# Autodesk Inventor assembly: Folded Door with the Rollers
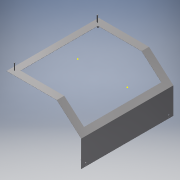
[picture p0: Inventor's stored thumbnail of the model, 180x180]
Saved by Autodesk Inventor 2016 (Build 200138000, 138)
## iProperties
Created: 2017-11-07
Part Number: Folded Door with the Rollers
Document SubType Name: Assembly
Designer: M227562
Author: M227562
## Documents named in this file (4)
- C:\Users\M227562\Documents\Arexu san\Folded Door with the Rollers.iam
- C:\Users\M227562\Documents\Arexu san\Lathe Cover\Folded in sheet metal\Part6.ipt
- C:\Users\M227562\Documents\Arexu san\L Braket for Wheels.ipt
- C:\Users\M227562\Documents\Arexu san\Door Carriage 2 Wheel EG7 with moving wheels.iam
## Components (7 placed, 3 different names)
1. Part6:1 — Rigid:1, Rigid:2, Rigid:5, Rigid:6
2. L Braket for Wheels:1 — Rigid:1, Rigid:3
3. L Braket for Wheels:2 — Rigid:2, Rigid:4
4. Door Carriage 2 Wheel EG7 with moving wheels:1 [sub-assembly] — Rigid:3
5. Door Carriage 2 Wheel EG7 with moving wheels:2 [sub-assembly] — Rigid:4
6. Door Carriage 2 Wheel EG7 with moving wheels:3 [sub-assembly] — Rigid:5
7. Door Carriage 2 Wheel EG7 with moving wheels:4 [sub-assembly] — Rigid:6
## Relationships (6: WeldJoint 6)
- Rigid:1 [WeldJoint]: Part6:1 ↔ L Braket for Wheels:1
- Rigid:2 [WeldJoint]: Part6:1 ↔ L Braket for Wheels:2
- Rigid:3 [WeldJoint]: L Braket for Wheels:1 ↔ Door Carriage 2 Wheel EG7 with moving wheels:1
- Rigid:4 [WeldJoint]: L Braket for Wheels:2 ↔ Door Carriage 2 Wheel EG7 with moving wheels:2
- Rigid:5 [WeldJoint] (-13 mm): Part6:1 ↔ Door Carriage 2 Wheel EG7 with moving wheels:3
- Rigid:6 [WeldJoint] (-13 mm): Part6:1 ↔ Door Carriage 2 Wheel EG7 with moving wheels:4
